# Autodesk Inventor assembly: support orangepi
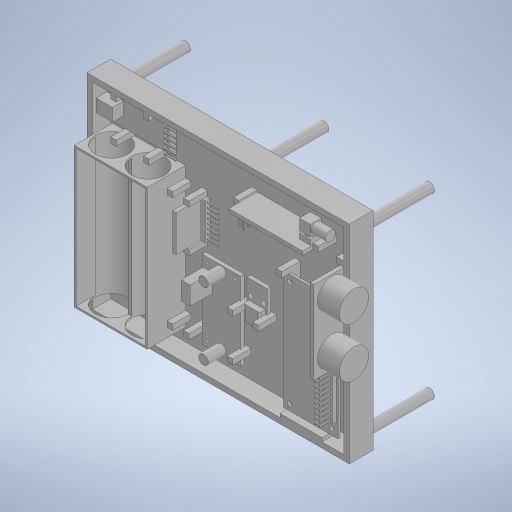
[picture p0: Inventor's stored thumbnail of the model, 512x512]
Saved by Autodesk Inventor 2024 (Build 280153000, 153)
## iProperties
Created: 2024-03-01
Part Number: support orangepi
Document SubType Name: Assembly
Designer: AdminForWorker
Title: support orangepi v17
Author: AdminForWorker
## Documents named in this file (10)
- C:\Users\phaly\Music\Perso\Projet voiture\3D\Support\support orangepi.iam
- C:\Users\phaly\Downloads\support orangepi v17\Component1.ipt
- C:\Users\phaly\Downloads\support orangepi v17\Component3.ipt
- C:\Users\phaly\Downloads\support orangepi v17\Component4.ipt
- C:\Users\phaly\Downloads\support orangepi v17\Component5.ipt
- C:\Users\phaly\Downloads\support orangepi v17\Component6.ipt
- C:\Users\phaly\Downloads\support orangepi v17\Component7.ipt
- C:\Users\phaly\Downloads\support orangepi v17\Component8.ipt
- C:\Users\phaly\Downloads\support orangepi v17\Component9.ipt
- C:\Users\phaly\Downloads\support orangepi v17\Component10.ipt
## Components (9 placed, 9 different names)
1. Component1:1 — Placage:7, Placage:8, Affleurement:1
2. Component3:1 — Placage:9, Affleurement:2, Placage:10
3. Component4:1 — Placage:11, Placage:12, Affleurement:3
4. Component5:1 — Placage:4, Placage:5, Placage:6
5. Component6:1 — Affleurement:4, Placage:13, Placage:14
6. Component7:1 — Placage:1, Placage:2, Placage:3, Placage:4, Placage:5, Placage:6, Placage:7, Placage:8, Affleurement:1, Placage:9, Affleurement:2, Placage:10, Placage:11, Placage:12, Affleurement:3, Affleurement:4, Placage:13, Placage:14
7. Component8:1 — Placage:1, Placage:2, Placage:3
8. Component9:1
9. Component10:1
## Relationships (18: Mate 14, Flush 4)
- Placage:1 [Mate]: Component7:1 ↔ Component8:1
- Placage:2 [Mate]: Component7:1 ↔ Component8:1
- Placage:3 [Mate]: Component7:1 ↔ Component8:1
- Placage:4 [Mate]: Component5:1 ↔ Component7:1
- Placage:5 [Mate]: Component5:1 ↔ Component7:1
- Placage:6 [Mate]: Component5:1 ↔ Component7:1
- Placage:7 [Mate]: Component1:1 ↔ Component7:1
- Placage:8 [Mate]: Component1:1 ↔ Component7:1
- Affleurement:1 [Flush]: Component1:1 ↔ Component7:1
- Placage:9 [Mate]: Component3:1 ↔ Component7:1
- Affleurement:2 [Flush]: Component3:1 ↔ Component7:1
- Placage:10 [Mate]: Component3:1 ↔ Component7:1
- Placage:11 [Mate]: Component4:1 ↔ Component7:1
- Placage:12 [Mate]: Component4:1 ↔ Component7:1
- Affleurement:3 [Flush]: Component4:1 ↔ Component7:1
- Affleurement:4 [Flush]: Component6:1 ↔ Component7:1
- Placage:13 [Mate]: Component6:1 ↔ Component7:1
- Placage:14 [Mate]: Component6:1 ↔ Component7:1
